# Autodesk Inventor assembly: reductor_12_10
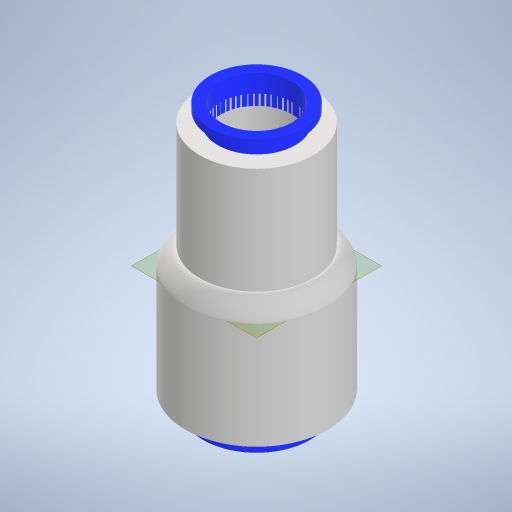
[picture p0: Inventor's stored thumbnail of the model, 512x512]
Saved by Autodesk Inventor 2024 (Build 280153000, 153)
## iProperties
Created: 2023-04-11
Part Number: reductor_12_10
Document SubType Name: Assembly
Designer: ferna
Author: ferna
## Documents named in this file (4)
- C:\Users\ferna\OneDrive - Universidad Católica de Chile\Bocas\RobotFlautista\Mold Design1\reductor_12_10.iam
- C:\Users\ferna\OneDrive - Universidad Católica de Chile\Bocas\RobotFlautista\entrada_manguera_2.ipt
- C:\Users\ferna\OneDrive - Universidad Católica de Chile\Bocas\RobotFlautista\reductor1210.ipt
- C:\Users\ferna\OneDrive - Universidad Católica de Chile\Bocas\RobotFlautista\entrada_manguera_2_big.ipt
## Components (3 placed, 3 different names)
1. entrada_manguera_2:1 — Mate:1, Mate:2
2. reductor1210:1 — Mate:1, Mate:2, Mate:3, Mate:4
3. entrada_manguera_2_big:1 — Mate:3, Mate:4
## Relationships (4: Mate 4)
- Mate:1 (-1.5 mm): entrada_manguera_2:1 ↔ reductor1210:1
- Mate:2: entrada_manguera_2:1 ↔ reductor1210:1
- Mate:3 (-1.5 mm): reductor1210:1 ↔ entrada_manguera_2_big:1
- Mate:4: reductor1210:1 ↔ entrada_manguera_2_big:1
